# Autodesk Inventor assembly: screwbase
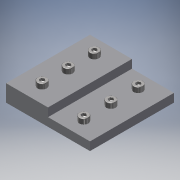
[picture p0: Inventor's stored thumbnail of the model, 180x180]
Saved by Autodesk Inventor 2019 (Build 230136000, 136)
## iProperties
Created: 2018-12-19
Part Number: screwbase
Document SubType Name: Assembly
Designer: assman
Author: assman
## Documents named in this file (4)
- D:\Inventor\CatFeeder\tests\screwbase.iam
- D:\Inventor\CatFeeder\tests\screwbase.ipt
- C:\Users\assman\Documents\Inventor\Content Center Files\R2019\en-US\DIN 912\DIN 912 - M3 x 0,5 x 10 x 8,75.ipt
- C:\Users\assman\Documents\Inventor\Content Center Files\R2019\en-US\DIN 912\DIN 912 - M3 x 0,5 x 5 x 3,75.ipt
## Components (7 placed, 3 different names)
1. screwbase:1 — Insert:1, Insert:2, Insert:3, Insert:4, Insert:5, Insert:6
2. DIN 912 - replaced by DIN EN ISO 4762 M3 x 10:1 — Insert:1
3. DIN 912 - replaced by DIN EN ISO 4762 M3 x 10:2 — Insert:2
4. DIN 912 - replaced by DIN EN ISO 4762 M3 x 10:3 — Insert:3
5. DIN 912 - replaced by DIN EN ISO 4762 M3 x 5:1 — Insert:4
6. DIN 912 - replaced by DIN EN ISO 4762 M3 x 5:2 — Insert:5
7. DIN 912 - replaced by DIN EN ISO 4762 M3 x 5:3 — Insert:6
## Relationships (6: Insert 6)
- Insert:1: screwbase:1 ↔ DIN 912 - replaced by DIN EN ISO 4762 M3 x 10:1
- Insert:2: screwbase:1 ↔ DIN 912 - replaced by DIN EN ISO 4762 M3 x 10:2
- Insert:3: screwbase:1 ↔ DIN 912 - replaced by DIN EN ISO 4762 M3 x 10:3
- Insert:4: screwbase:1 ↔ DIN 912 - replaced by DIN EN ISO 4762 M3 x 5:1
- Insert:5: screwbase:1 ↔ DIN 912 - replaced by DIN EN ISO 4762 M3 x 5:2
- Insert:6: screwbase:1 ↔ DIN 912 - replaced by DIN EN ISO 4762 M3 x 5:3
